# Autodesk Inventor assembly: ConjuntoSoporteMangueras
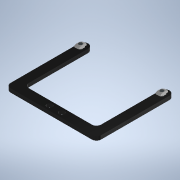
[picture p0: Inventor's stored thumbnail of the model, 180x180]
Saved by Autodesk Inventor 2020.2 (Build 242310000, 310)
## iProperties
Created: 2021-03-01
Part Number: ConjuntoSoporteMangueras
Document SubType Name: Assembly
Designer: JK
Author: JK
## Documents named in this file (4)
- C:\Users\JK\Documents\Inventor\BioMixer\DispensadorPolvo\ConjuntoSoporteMangueras.iam
- C:\Users\JK\Documents\Inventor\BioMixer\SoporteMangueras.ipt
- C:\Users\JK\Documents\Inventor\BioMixer\PernoM5x10Plano.ipt
- C:\Users\JK\Documents\Inventor\BioMixer\TuercaTM5Perfil2020.ipt
## Components (5 placed, 3 different names)
1. SoporteMangueras:1 — Mate:1, Mate:2, Mate:3, Angle:2, Mate:6
2. PernoM5x10Plano:1 — Mate:2, Flush:1, Mate:3, Mate:4
3. PernoM5x10Plano:2 — Mate:1, Flush:1, Mate:5
4. TuercaTM5Perfil2020:1 — Mate:5, Angle:1, Flush:2
5. TuercaTM5Perfil2020:2 — Mate:4, Angle:1, Angle:2, Flush:2, Mate:6
## Relationships (10: Mate 6, Flush 2, Angle 2)
- Mate:1: SoporteMangueras:1 ↔ PernoM5x10Plano:2
- Mate:2: SoporteMangueras:1 ↔ PernoM5x10Plano:1
- Flush:1: PernoM5x10Plano:1 ↔ PernoM5x10Plano:2
- Mate:3: SoporteMangueras:1 ↔ PernoM5x10Plano:1
- Mate:4: PernoM5x10Plano:1 ↔ TuercaTM5Perfil2020:2
- Mate:5: PernoM5x10Plano:2 ↔ TuercaTM5Perfil2020:1
- Angle:1 (0 deg): TuercaTM5Perfil2020:1 ↔ TuercaTM5Perfil2020:2
- Angle:2 (0 deg): SoporteMangueras:1 ↔ TuercaTM5Perfil2020:2
- Flush:2: TuercaTM5Perfil2020:1 ↔ TuercaTM5Perfil2020:2
- Mate:6 (0.5 mm): SoporteMangueras:1 ↔ TuercaTM5Perfil2020:2
